# Autodesk Inventor assembly: Half overlay hinge for aluminium frame
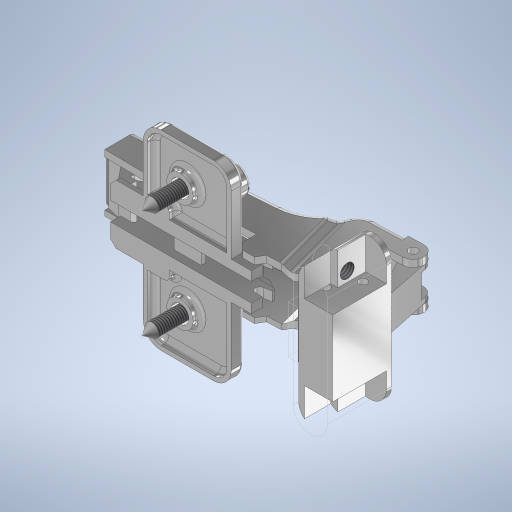
[picture p0: Inventor's stored thumbnail of the model, 512x512]
Saved by Autodesk Inventor 2024 (Build 280153000, 153)
## iProperties
Created: 2014-01-06
Part Number: Half overlay hinge for aluminium frame
Document SubType Name: Assembly
Designer: G. Kazokaitis
Author: G. Kazokaitis
## Documents named in this file (7)
- C:\W4INV 2024 Design\_LIBRARY\Hinges\HINGE FOR ALUMINIUM FRAME\Half overlay hinge for aluminium frame.iam
- C:\W4INV 2024 Design\LIBRARY\Hinges\Parts\Hinge for aluminium frame\Half overlay case.ipt
- C:\W4INV 2024 Design\LIBRARY\Hinges\Parts\Hinge for aluminium frame\Lever for half overlay hinge.ipt
- C:\W4INV 2024 Design\LIBRARY\Hinges\Parts\Hinge for aluminium frame\Linkage for half overlay hinge.ipt
- C:\W4INV 2024 Design\LIBRARY\Hinges\Parts\Hinge for aluminium frame\Mounting plate.ipt
- C:\W4INV 2024 Design\LIBRARY\Hinges\Parts\Hinge for aluminium frame\Cup.ipt
- C:\W4INV 2024 Design\LIBRARY\Hinges\HINGE FOR ALUMINIUM FRAME.iam
## Components (5 placed, 5 different names)
1. Mounting plate:1 — Flush:1, Flush:2, Mate:1, Flush:4, Mate:11, Mate:12
2. Cup:1 — Mate:17, Mate:18, Mate:19, Half overlay opening angle
3. Half overlay case:1 — Flush:4, Mate:11, Mate:12, Mate:13, Mate:14, Mate:15, Mate:16, Half overlay opening angle
4. Lever for half overlay hinge:1 — Mate:13, Mate:14, Mate:17, Mate:19
5. Linkage for half overlay hinge:1 — Mate:15, Mate:16, Mate:18
## Relationships (14: Mate 10, Flush 3, Angle 1)
- Flush:1: Mounting plate:1
- Flush:2: Mounting plate:1
- Mate:1: Mounting plate:1
- Flush:4: Mounting plate:1 ↔ Half overlay case:1
- Mate:11: Mounting plate:1 ↔ Half overlay case:1
- Mate:12: Mounting plate:1 ↔ Half overlay case:1
- Mate:13: Half overlay case:1 ↔ Lever for half overlay hinge:1
- Mate:14: Half overlay case:1 ↔ Lever for half overlay hinge:1
- Mate:15: Half overlay case:1 ↔ Linkage for half overlay hinge:1
- Mate:16: Half overlay case:1 ↔ Linkage for half overlay hinge:1
- Mate:17: Cup:1 ↔ Lever for half overlay hinge:1
- Mate:18: Cup:1 ↔ Linkage for half overlay hinge:1
- Mate:19 (1.9 mm): Cup:1 ↔ Lever for half overlay hinge:1
- Half overlay opening angle [Angle] (180 deg): Cup:1 ↔ Half overlay case:1
## Named parameters: Offset_distance = 37 mm
